# Autodesk Inventor assembly: furnace1
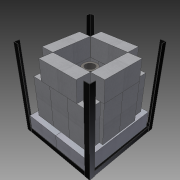
[picture p0: Inventor's stored thumbnail of the model, 180x180]
Saved by Autodesk Inventor 2015 (Build 190159000, 159)
## iProperties
Created: 2017-03-31
Part Number: furnace1
Document SubType Name: Assembly
Designer: miki
Author: miki
## Documents named in this file (7)
- V:\DATA\PROJECT\electric_furnace\inventor\furnace1.iam
- V:\DATA\PROJECT\electric_furnace\inventor\Katownik_stalowy_45cm.ipt
- V:\DATA\PROJECT\electric_furnace\inventor\IFB-23.ipt
- V:\DATA\PROJECT\electric_furnace\inventor\Katownik_stalowy_50cm.ipt
- V:\DATA\PROJECT\electric_furnace\inventor\Termalica_60x20x10cm.ipt
- V:\DATA\PROJECT\electric_furnace\inventor\Tygiel_TG5.ipt
- V:\DATA\PROJECT\electric_furnace\inventor\cast_hand.ipt
## Components (28 placed, 6 different names)
1. Tygiel_TG5:1
2. cast_hand:1
3. Katownik_stalowy_50cm:1 — Flush:6, Flush:8, Flush:11
4. Katownik_stalowy_45cm:2 — Flush:2, Flush:4
5. Katownik_stalowy_45cm:3 — Flush:1, Flush:3
6. Katownik_stalowy_45cm:4 — Flush:1, Flush:3
7. Katownik_stalowy_50cm:2 — Flush:7, Flush:10, Flush:11
8. Katownik_stalowy_50cm:3 — Flush:5, Flush:6, Flush:7, Flush:8, Flush:9
9. Katownik_stalowy_50cm:4 — Flush:5, Flush:9, Flush:10
10. Katownik_stalowy_45cm:1 — Flush:2, Flush:4
11. Termalica_60x20x10cm:1 — Mate:1, Flush:12, Flush:13, Mate:2, Mate:3, Mate:5
12. Termalica_60x20x10cm:2 — Mate:1, Flush:12, Flush:13, Mate:4, Mate:6
13. IFB-23:1 — Mate:2, Rigid:1
14. IFB-23:2 — Rigid:1
15. IFB-23:4 — Mate:7
16. IFB-23:8 — Rigid:2
17. IFB-23:9 — Rigid:2, Mate:3, Mate:10
18. IFB-23:10 — Mate:9
19. IFB-23:11 — Mate:4
20. IFB-23:12 — Mate:5
21. IFB-23:13 — Rigid:5, Mate:7
22. IFB-23:14 — Rigid:5
23. IFB-23:15
24. IFB-23:16 — Mate:8
25. IFB-23:17 — Mate:6
26. IFB-23:18 — Mate:8
27. IFB-23:19 — Mate:9
28. IFB-23:20 — Mate:10
## Relationships (30: Flush 13, Mate 10, WeldJoint 7)
- Flush:1: Katownik_stalowy_45cm:3 ↔ Katownik_stalowy_45cm:4
- Flush:2: Katownik_stalowy_45cm:2 ↔ Katownik_stalowy_45cm:1
- Flush:3: Katownik_stalowy_45cm:3 ↔ Katownik_stalowy_45cm:4
- Flush:4: Katownik_stalowy_45cm:2 ↔ Katownik_stalowy_45cm:1
- Flush:5: Katownik_stalowy_50cm:3 ↔ Katownik_stalowy_50cm:4
- Flush:6: Katownik_stalowy_50cm:1 ↔ Katownik_stalowy_50cm:3
- Flush:7: Katownik_stalowy_50cm:2 ↔ Katownik_stalowy_50cm:3
- Flush:8: Katownik_stalowy_50cm:1 ↔ Katownik_stalowy_50cm:3
- Flush:9: Katownik_stalowy_50cm:3 ↔ Katownik_stalowy_50cm:4
- Flush:10: Katownik_stalowy_50cm:2 ↔ Katownik_stalowy_50cm:4
- Flush:11: Katownik_stalowy_50cm:1 ↔ Katownik_stalowy_50cm:2
- Mate:1: Termalica_60x20x10cm:1 ↔ Termalica_60x20x10cm:2
- Flush:12: Termalica_60x20x10cm:1 ↔ Termalica_60x20x10cm:2
- Flush:13: Termalica_60x20x10cm:1 ↔ Termalica_60x20x10cm:2
- Mate:2: Termalica_60x20x10cm:1 ↔ IFB-23:1
- Rigid:1 [WeldJoint]: IFB-23:1 ↔ IFB-23:2
- Rigid:2 [WeldJoint]: IFB-23:8 ↔ IFB-23:9
- Mate:3: Termalica_60x20x10cm:1 ↔ IFB-23:9
- [WeldJoint]: IFB-23:10 ↔ IFB-23:11
- Mate:4: Termalica_60x20x10cm:2 ↔ IFB-23:11
- [WeldJoint]: IFB-23:12 ↔ IFB-23:13
- Rigid:5 [WeldJoint]: IFB-23:13 ↔ IFB-23:14
- Mate:5: Termalica_60x20x10cm:1 ↔ IFB-23:12
- [WeldJoint]: IFB-23:15 ↔ IFB-23:16
- [WeldJoint]: IFB-23:16 ↔ IFB-23:17
- Mate:6: Termalica_60x20x10cm:2 ↔ IFB-23:17
- Mate:7: IFB-23:4 ↔ IFB-23:13
- Mate:8: IFB-23:16 ↔ IFB-23:18
- Mate:9: IFB-23:10 ↔ IFB-23:19
- Mate:10: IFB-23:9 ↔ IFB-23:20
## Named parameters: d19_d16 = 0 mm, d21_d16 = 0 mm, d24_d21_d16 = 0 mm, d25_d22 = 0 mm
